# Autodesk Inventor assembly: Rover
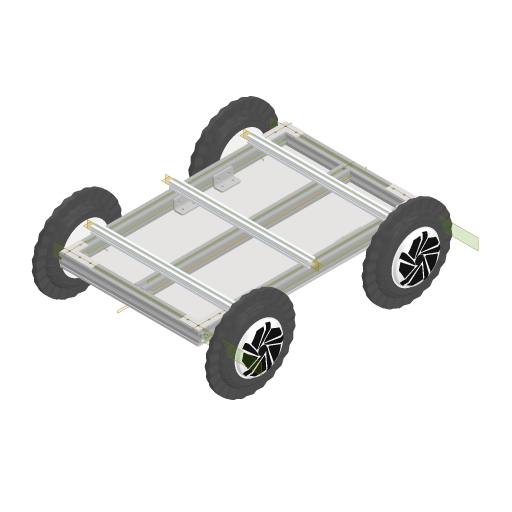
[picture p0: Inventor's stored thumbnail of the model, 512x512]
Saved by Autodesk Inventor 2023.2 (Build 272271030, 271C)
## iProperties
Created: 2024-10-30
Part Number: Rover
Document SubType Name: Assembly
Designer: I9232
Author: I9232
## Documents named in this file (10)
- D:\!Rover\Rover\Rover_construction\Rover.iam
- D:\!Rover\Rover\Rover_construction\platform.ipt
- D:\!Rover\Rover\Rover_construction\Motor, BLDC, Hoverboard Wheel, 8.0in.ipt
- D:\!Rover\Rover\Rover_construction\Деталь14.ipt
- D:\!Rover\Rover\Rover_construction\Profil 20x20.ipt
- D:\!Rover\Rover\Rover_construction\Крепление мотора.iam
- D:\!Rover\Rover\Rover_construction\Copter.ipt
- D:\!Rover\Rover\Rover_construction\Korpus.ipt
- D:\!Rover\Rover\Rover_construction\Уголок для профиля\Уголок для профиля.ipt
- D:\!Rover\Rover\Rover_construction\5f9134727ab186bd9543c462de202546\5f9134727ab186bd9543c462de202546.ipt
## Components (27 placed, 10 different names)
1. platform:1 — Совмещение:1, Совмещение:2, Совмещение:3, Совмещение:4, Совмещение:14, Совмещение:15, Совмещение:54, Совмещение:55, Совмещение:56, Совмещение:59, Совмещение:61, Совмещение:62, Совмещение:107, Совмещение:119, Совмещение:120, Совмещение:121, Совмещение:140, Совмещение:141, Совмещение:142, Совмещение:143
2. Copter:1
3. Korpus:1
4. Мотор гироскутера — Совмещение:122, Совмещение:123, Совмещение:124
5. Motor, BLDC, Hoverboard Wheel, 8.0in:4 — Совмещение:116, Совмещение:117, Совмещение:118
6. Motor, BLDC, Hoverboard Wheel, 8.0in:5 — Совмещение:112, Совмещение:113, Совмещение:115
7. Motor, BLDC, Hoverboard Wheel, 8.0in:6 — Совмещение:110, Совмещение:111, Совмещение:114
8. Profil 20x20:1 — Совмещение:24, Совмещение:25, Совмещение:128, Симметрия:3, Совмещение:129
9. Profil 20x20:2 — Совмещение:20, Совмещение:21, Совмещение:127, Симметрия:3
10. Profil 20x20:3 — Совмещение:22, Совмещение:23
11. профиль 30x30:3 — Совмещение:3, Совмещение:15, Совмещение:20, Совмещение:21, Совмещение:22, Совмещение:23, Совмещение:24, Совмещение:25, Совмещение:92, Совмещение:125, Совмещение:126, Совмещение:131, Заподлицо:4, Заподлицо:6, Совмещение:144, Совмещение:145
12. профиль 30x30:4 — Совмещение:4, Совмещение:14, Совмещение:60, Заподлицо:1, Заподлицо:2, Совмещение:130, Совмещение:138, Совмещение:139, Совмещение:146, Совмещение:147
13. профиль 30x30:5 — Совмещение:55, Совмещение:59, Совмещение:63, Совмещение:92, Совмещение:131, Совмещение:133, Совмещение:134, Совмещение:136, Совмещение:137
14. профиль 30x30:6 — Совмещение:54, Совмещение:56, Совмещение:60, Совмещение:129, Совмещение:130, Совмещение:132, Совмещение:135, Заподлицо:3, Заподлицо:5
15. профиль 30x30:7 — Совмещение:61, Совмещение:62, Совмещение:63
16. Крепление мотора:1 [sub-assembly] — Совмещение:116, Совмещение:117, Совмещение:118, Совмещение:119, Заподлицо:1, Симметрия:2
17. Крепление мотора:2 [sub-assembly] — Совмещение:107, Совмещение:122, Совмещение:123, Совмещение:124, Совмещение:125, Симметрия:2, Совмещение:128
18. Крепление мотора:3 [sub-assembly] — Совмещение:110, Совмещение:111, Совмещение:114, Совмещение:121, Заподлицо:2, Симметрия:1
19. Крепление мотора:4 [sub-assembly] — Совмещение:112, Совмещение:113, Совмещение:115, Совмещение:120, Совмещение:126, Симметрия:1, Совмещение:127
20. Уголок для профиля:1 — Совмещение:132, Заподлицо:4, Заподлицо:5
21. Уголок для профиля:2 — Совмещение:133, Совмещение:137, Совмещение:138
22. Уголок для профиля:3 — Совмещение:135, Заподлицо:3, Совмещение:139
23. Уголок для профиля:4 — Совмещение:134, Совмещение:136, Заподлицо:6
24. 5f9134727ab186bd9543c462de202546:1 — Совмещение:140, Совмещение:146
25. 5f9134727ab186bd9543c462de202546:2 — Совмещение:141, Совмещение:147
26. 5f9134727ab186bd9543c462de202546:3 — Совмещение:142, Совмещение:145
27. 5f9134727ab186bd9543c462de202546:4 — Совмещение:143, Совмещение:144
## Relationships (69: Mate 60, Flush 6, Symmetry 3)
- Совмещение:1 [Mate]: platform:1
- Совмещение:2 [Mate]: platform:1
- Совмещение:3 [Mate]: platform:1 ↔ профиль 30x30:3
- Совмещение:4 [Mate]: platform:1 ↔ профиль 30x30:4
- Совмещение:14 [Mate]: platform:1 ↔ профиль 30x30:4
- Совмещение:15 [Mate]: platform:1 ↔ профиль 30x30:3
- Совмещение:20 [Mate]: Profil 20x20:2 ↔ профиль 30x30:3
- Совмещение:21 [Mate]: Profil 20x20:2 ↔ профиль 30x30:3
- Совмещение:22 [Mate]: Profil 20x20:3 ↔ профиль 30x30:3
- Совмещение:23 [Mate]: Profil 20x20:3 ↔ профиль 30x30:3
- Совмещение:24 [Mate]: Profil 20x20:1 ↔ профиль 30x30:3
- Совмещение:25 [Mate]: Profil 20x20:1 ↔ профиль 30x30:3
- Совмещение:54 [Mate]: platform:1 ↔ профиль 30x30:6
- Совмещение:55 [Mate]: platform:1 ↔ профиль 30x30:5
- Совмещение:56 [Mate]: platform:1 ↔ профиль 30x30:6
- Совмещение:59 [Mate]: platform:1 ↔ профиль 30x30:5
- Совмещение:60 [Mate]: профиль 30x30:4 ↔ профиль 30x30:6
- Совмещение:61 [Mate]: platform:1 ↔ профиль 30x30:7
- Совмещение:62 [Mate]: platform:1 ↔ профиль 30x30:7
- Совмещение:63 [Mate]: профиль 30x30:5 ↔ профиль 30x30:7
- Совмещение:92 [Mate]: профиль 30x30:3 ↔ профиль 30x30:5
- Совмещение:107 [Mate]: platform:1 ↔ Крепление мотора:2
- Совмещение:110 [Mate]: Motor, BLDC, Hoverboard Wheel, 8.0in:6 ↔ Крепление мотора:3
- Совмещение:111 [Mate]: Motor, BLDC, Hoverboard Wheel, 8.0in:6 ↔ Крепление мотора:3
- Совмещение:112 [Mate]: Motor, BLDC, Hoverboard Wheel, 8.0in:5 ↔ Крепление мотора:4
- Совмещение:113 [Mate]: Motor, BLDC, Hoverboard Wheel, 8.0in:5 ↔ Крепление мотора:4
- Совмещение:114 [Mate]: Motor, BLDC, Hoverboard Wheel, 8.0in:6 ↔ Крепление мотора:3
- Совмещение:115 [Mate]: Motor, BLDC, Hoverboard Wheel, 8.0in:5 ↔ Крепление мотора:4
- Совмещение:116 [Mate]: Motor, BLDC, Hoverboard Wheel, 8.0in:4 ↔ Крепление мотора:1
- Совмещение:117 [Mate]: Motor, BLDC, Hoverboard Wheel, 8.0in:4 ↔ Крепление мотора:1
- Совмещение:118 [Mate]: Motor, BLDC, Hoverboard Wheel, 8.0in:4 ↔ Крепление мотора:1
- Совмещение:119 [Mate]: platform:1 ↔ Крепление мотора:1
- Совмещение:120 [Mate]: platform:1 ↔ Крепление мотора:4
- Совмещение:121 [Mate]: platform:1 ↔ Крепление мотора:3
- Заподлицо:1 [Flush]: профиль 30x30:4 ↔ Крепление мотора:1
- Совмещение:122 [Mate]: Мотор гироскутера ↔ Крепление мотора:2
- Совмещение:123 [Mate]: Мотор гироскутера ↔ Крепление мотора:2
- Совмещение:124 [Mate]: Мотор гироскутера ↔ Крепление мотора:2
- Совмещение:125 [Mate]: профиль 30x30:3 ↔ Крепление мотора:2
- Заподлицо:2 [Flush]: профиль 30x30:4 ↔ Крепление мотора:3
- Совмещение:126 [Mate]: профиль 30x30:3 ↔ Крепление мотора:4
- Симметрия:1 [Symmetry]: Крепление мотора:3 ↔ Крепление мотора:4
- Симметрия:2 [Symmetry]: Крепление мотора:1 ↔ Крепление мотора:2
- Совмещение:127 [Mate]: Profil 20x20:2 ↔ Крепление мотора:4
- Совмещение:128 [Mate]: Profil 20x20:1 ↔ Крепление мотора:2
- Симметрия:3 [Symmetry]: Profil 20x20:1 ↔ Profil 20x20:2
- Совмещение:129 [Mate] (85.251 mm): Profil 20x20:1 ↔ профиль 30x30:6
- Совмещение:130 [Mate]: профиль 30x30:4 ↔ профиль 30x30:6
- Совмещение:131 [Mate]: профиль 30x30:3 ↔ профиль 30x30:5
- Совмещение:132 [Mate]: профиль 30x30:6 ↔ Уголок для профиля:1
- Совмещение:133 [Mate]: профиль 30x30:5 ↔ Уголок для профиля:2
- Совмещение:134 [Mate]: профиль 30x30:5 ↔ Уголок для профиля:4
- Совмещение:135 [Mate]: профиль 30x30:6 ↔ Уголок для профиля:3
- Заподлицо:3 [Flush]: профиль 30x30:6 ↔ Уголок для профиля:3
- Заподлицо:4 [Flush]: профиль 30x30:3 ↔ Уголок для профиля:1
- Заподлицо:5 [Flush]: профиль 30x30:6 ↔ Уголок для профиля:1
- Совмещение:136 [Mate]: профиль 30x30:5 ↔ Уголок для профиля:4
- Заподлицо:6 [Flush]: профиль 30x30:3 ↔ Уголок для профиля:4
- Совмещение:137 [Mate]: профиль 30x30:5 ↔ Уголок для профиля:2
- Совмещение:138 [Mate]: профиль 30x30:4 ↔ Уголок для профиля:2
- Совмещение:139 [Mate]: профиль 30x30:4 ↔ Уголок для профиля:3
- Совмещение:140 [Mate]: platform:1 ↔ 5f9134727ab186bd9543c462de202546:1
- Совмещение:141 [Mate]: platform:1 ↔ 5f9134727ab186bd9543c462de202546:2
- Совмещение:142 [Mate]: platform:1 ↔ 5f9134727ab186bd9543c462de202546:3
- Совмещение:143 [Mate]: platform:1 ↔ 5f9134727ab186bd9543c462de202546:4
- Совмещение:144 [Mate]: профиль 30x30:3 ↔ 5f9134727ab186bd9543c462de202546:4
- Совмещение:145 [Mate]: профиль 30x30:3 ↔ 5f9134727ab186bd9543c462de202546:3
- Совмещение:146 [Mate]: профиль 30x30:4 ↔ 5f9134727ab186bd9543c462de202546:1
- Совмещение:147 [Mate]: профиль 30x30:4 ↔ 5f9134727ab186bd9543c462de202546:2
